# Autodesk Inventor assembly: リンク_6_1
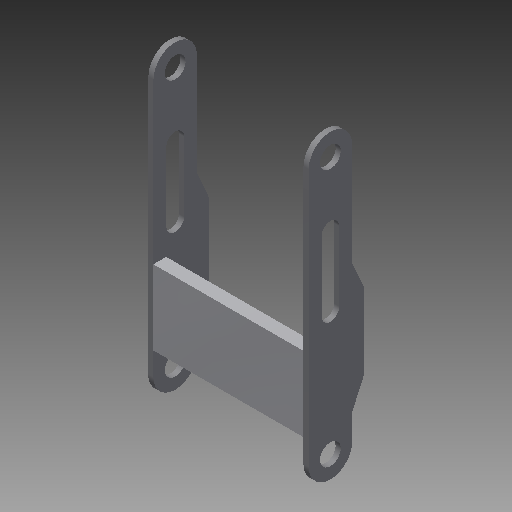
[picture p0: Inventor's stored thumbnail of the model, 512x512]
Saved by Autodesk Inventor 2018 (Build 220112000, 112)
## iProperties
Created: 2016-08-23
Part Number: リンク_6_1
Material: 一般
Document SubType Name: Assembly
Designer: hiro
Mass: 25.265 g
Surface Area: 146.992 cm^2
Volume: 11.3922 cm^3
Density: 2.21774 g/cm^3
Author: hiro
## Documents named in this file (3)
- Z:\OPR\OpenPlatform_ver1_0\下半身_160823\リンク\リンク_6_3.iam
- Z:\OPR\OpenPlatform_ver1_0\下半身\リンク\ふくらはぎ\リンク_ふくらはぎ_サブフレーム_1_2(予備案).ipt
- Z:\OPR\OpenPlatform_ver1_0\下半身_160823\リンク\リンク_メインフレーム_6_1.ipt
## Components (3 placed, 2 different names)
1. リンク_ふくらはぎ_サブフレーム_1_2(予備案):1 — 挿入:25, 挿入:26, 挿入:27, 挿入:30, 挿入:31, 挿入:32
2. リンク_メインフレーム_6_1:1 — 挿入:30, 挿入:31, 挿入:32
3. リンク_メインフレーム_6_1:2 — 挿入:25, 挿入:26, 挿入:27
## Relationships (6: Insert 6)
- 挿入:25 [Insert]: リンク_ふくらはぎ_サブフレーム_1_2(予備案):1 ↔ リンク_メインフレーム_6_1:2
- 挿入:26 [Insert]: リンク_ふくらはぎ_サブフレーム_1_2(予備案):1 ↔ リンク_メインフレーム_6_1:2
- 挿入:27 [Insert]: リンク_ふくらはぎ_サブフレーム_1_2(予備案):1 ↔ リンク_メインフレーム_6_1:2
- 挿入:30 [Insert]: リンク_ふくらはぎ_サブフレーム_1_2(予備案):1 ↔ リンク_メインフレーム_6_1:1
- 挿入:31 [Insert]: リンク_ふくらはぎ_サブフレーム_1_2(予備案):1 ↔ リンク_メインフレーム_6_1:1
- 挿入:32 [Insert]: リンク_ふくらはぎ_サブフレーム_1_2(予備案):1 ↔ リンク_メインフレーム_6_1:1
